# Autodesk Inventor assembly: pivot
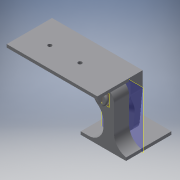
[picture p0: Inventor's stored thumbnail of the model, 180x180]
Saved by Autodesk Inventor 2019 (Build 230136000, 136)
## iProperties
Created: 2019-02-28
Part Number: pivot
Document SubType Name: Assembly
Designer: erwin
Author: erwin
## Documents named in this file (3)
- D:\GitHub\DrowningWarnings\wave_simulator\pivot.iam
- D:\GitHub\DrowningWarnings\wave_simulator\pivotholder.ipt
- D:\GitHub\DrowningWarnings\model\pivot2.ipt
## Components (2 placed, 2 different names)
1. pivotholder:1 — Flush:1, Flush:2
2. pivot2:1 — Flush:1, Flush:2
## Relationships (2: Flush 2)
- Flush:1: pivotholder:1 ↔ pivot2:1
- Flush:2: pivotholder:1 ↔ pivot2:1
